# Autodesk Inventor assembly: CATFEEDER
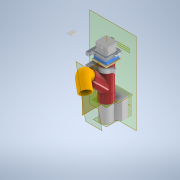
[picture p0: Inventor's stored thumbnail of the model, 180x180]
Saved by Autodesk Inventor 2020.5 (Build 245400000, 400)
## iProperties
Created: 2022-02-21
Part Number: CATFEEDER
Document SubType Name: Assembly
Designer: EDDY
Author: EDDY
## iProperties of the stored document CTF_beugel v1.ipt
Created: 2022-02-21
Part Number: CTF_beugel
Material: Generic
Document SubType Name: Modeling
Designer: Administrator
Density: 1 g/cm^3
Appearance: Default
Sending System: Autodesk Inventor 2021
Title: CTF_beugel v1
Author: Administrator
## iProperties of the stored document CTF_SUPPORTKLEMSPLITBUIS v1.ipt
Created: 2022-02-21
Part Number: CTF_SUPPORTKLEMSPLITBUIS
Material: Generic
Document SubType Name: Modeling
Designer: Administrator
Density: 1 g/cm^3
Appearance: Default
Sending System: Autodesk Inventor 2021
Title: CTF_SUPPORTKLEMSPLITBUIS v1
Author: Administrator
## iProperties of the stored document CFT_NEMA17 17HS4401 v12.ipt
Created: 2022-03-18
Part Number: CFT_NEMA17  17HS4401
Material: Generic
Document SubType Name: Modeling
Designer: Administrator
Density: 1 g/cm^3
Appearance: Default
Sending System: Autodesk Inventor 2021
Title: CFT_NEMA17 17HS4401 v12
Author: Administrator
## iProperties of the stored document CTF_MOTORFLENS v14.ipt
Created: 2022-02-21
Part Number: CTF_MOTORFLENS
Material: Generic
Document SubType Name: Modeling
Designer: Administrator
Density: 1 g/cm^3
Appearance: Default
Sending System: Autodesk Inventor 2021
Title: CTF_MOTORFLENS v14
Author: Administrator
## iProperties of the stored document CFT_arhimedes v20.ipt
Created: 2022-02-21
Part Number: CFT_arhimedes
Material: Generic
Document SubType Name: Modeling
Designer: Administrator
Density: 1 g/cm^3
Appearance: Default
Sending System: Autodesk Inventor 2021
Title: CFT_arhimedes v20
Author: Administrator
## iProperties of the stored document CTF_motortussenflens v5.ipt
Created: 2022-02-21
Part Number: CTF_motortussenflens
Material: Generic
Document SubType Name: Modeling
Designer: Administrator
Density: 1 g/cm^3
Appearance: Default
Sending System: Autodesk Inventor 2021
Title: CTF_motortussenflens v5
Author: Administrator
## iProperties of the stored document CTF_ELLEBOOG90 v6.ipt
Created: 2022-02-21
Part Number: CTF_ELLEBOOG90
Material: Generic
Document SubType Name: Modeling
Designer: Administrator
Density: 1 g/cm^3
Appearance: Default
Sending System: Autodesk Inventor 2021
Title: CTF_ELLEBOOG90 v6
Author: Administrator
## iProperties of the stored document CTF_SPLTSTUK v11.ipt
Created: 2022-02-21
Part Number: CTF_SPLTSTUK
Material: Generic
Document SubType Name: Modeling
Designer: Administrator
Density: 1 g/cm^3
Appearance: Default
Sending System: Autodesk Inventor 2021
Title: CTF_SPLTSTUK v11
Author: Administrator
## Documents named in this file (25)
- C:\IV2020_DATA\IV2020_CADFILES\Catfeeder\CATFEEDER.iam
- **C:\IV2020_DATA\IV2020_CADFILES\Catfeeder\CATFEEDER.iam*LocalDocs*xAaaaabaaAaaaaaaaAaaaa2dnAh*CTF_MOTORFLENS v14.ipt
- **C:\IV2020_DATA\IV2020_CADFILES\Catfeeder\CATFEEDER.iam*LocalDocs*xAaaaanaaAaaaaaaaAaaaqlbl5b*CTF_motortussenflens v5.ipt
- **C:\IV2020_DATA\IV2020_CADFILES\Catfeeder\CATFEEDER.iam*LocalDocs*xAaaaapaaAaaaaaaaAaaaqkmmNf*CFT_arhimedes v20.ipt
- **C:\IV2020_DATA\IV2020_CADFILES\Catfeeder\CATFEEDER.iam*LocalDocs*xAaaaqibaAaaaaaaaAaaaqnyw4c*CTF_ELLEBOOG90 v6.ipt
- **C:\IV2020_DATA\IV2020_CADFILES\Catfeeder\CATFEEDER.iam*LocalDocs*xAaaaaaaaAaaaaaaaAaaaaebq2g*CTF_SUPPORTKLEMSPLITBUIS v1.ipt
- **C:\IV2020_DATA\IV2020_CADFILES\Catfeeder\CATFEEDER.iam*LocalDocs*xAaaaahcaAaaaaaaaAaaaakzuIb*CTF_beugel v1.ipt
- **C:\IV2020_DATA\IV2020_CADFILES\Catfeeder\CATFEEDER.iam*LocalDocs*xAaaaqzbaAaaaaaaaAaaaqedeCa*CTF_SPLTSTUK v11.ipt
- C:\IV2020_DATA\IV2020_CADFILES\Imported Components\CTF_steunmotor\CTF_steunmotor.ipt
- C:\IV2020_DATA\IV2020_CADFILES\Imported Components\CFT_motorklem\CFT_motorklem.ipt
- C:\IV2020_DATA\IV2020_CADFILES\Catfeeder\CFT_kast.ipt
- C:\IV2020_DATA\IV2020_CADFILES\Catfeeder\CFT_koppelstuk.ipt
- C:\IV2020_DATA\IV2020_CADFILES\Imported Components\Stepper_Driver_WINOMO_DRV8825_RP_A4988\Stepper_Driver_WINOMO_DRV8825_RP_A4988.ipt
- **C:\IV2020_DATA\IV2020_CADFILES\Catfeeder\CATFEEDER.iam*LocalDocs*xAaaaa0caAaaaaaaaAaaaq4zbYa*CFT_NEMA17 17HS4401 v12.ipt
- C:\IV2020_DATA\IV2020_CADFILES\Catfeeder\Archimedes2schroef.ipt
- C:\IV2020_DATA\IV2020_CADFILES\Catfeeder\CTF_GOOT.ipt
- C:\IV2020_DATA\IV2020_CADFILES\Catfeeder\CTF_deksel.ipt
- C:\IV2020_DATA\IV2020_CADFILES\Catfeeder\CTF_MOTORFLENS v14.ipt
- C:\IV2020_DATA\IV2020_CADFILES\Catfeeder\CTF_motortussenflens v5.ipt
- C:\IV2020_DATA\IV2020_CADFILES\Catfeeder\CFT_arhimedes v20.ipt
- C:\IV2020_DATA\IV2020_CADFILES\Catfeeder\CTF_ELLEBOOG90 v6.ipt
- C:\IV2020_DATA\IV2020_CADFILES\Catfeeder\CTF_SUPPORTKLEMSPLITBUIS v1.ipt
- C:\IV2020_DATA\IV2020_CADFILES\Catfeeder\CTF_beugel v1.ipt
- C:\IV2020_DATA\IV2020_CADFILES\Catfeeder\CTF_SPLTSTUK v11.ipt
- C:\IV2020_DATA\IV2020_CADFILES\Catfeeder\CFT_NEMA17 17HS4401 v12.ipt
## Components (21 placed, 16 different names)
1. CTF_MOTORFLENS v14:1 — Mate:1, Mate:2, Angle:1, Mate:4, Angle:3, Angle:5, Mate:9, Mate:12, Mate:19, Flush:4
2. CTF_motortussenflens v5:1 — Mate:1, Mate:2, Angle:1, Mate:4, Insert:3, Mate:13, Mate:15, Flush:5, Mate:32
3. CFT_arhimedes v20:1 — Insert:3, Mate:31
4. CTF_ELLEBOOG90 v6:1 — Angle:3, Flush:1, Mate:18, Mate:27, Mate:28, Mate:29, Mate:30
5. CTF_ELLEBOOG90 v6:2 — Angle:6, Mate:10, Mate:11
6. CTF_SUPPORTKLEMSPLITBUIS v1:1 — Angle:5, Mate:7, Mate:8, Mate:19, Flush:3, Flush:6, Flush:7
7. CTF_beugel v1:1 — Mate:7, Mate:8
8. CTF_SPLTSTUK v11:1 — Mate:9, Angle:6, Flush:1, Mate:10, Mate:11, Mate:12, Mate:17, Mate:28, Mate:30, Flush:10, Flush:11, Flush:12, Flush:13, Flush:19, Flush:20
9. CTF_steunmotor:1 — Mate:13, Mate:15, Mate:16, Angle:7, Mate:23, Angle:8
10. CFT_motorklem:1 — Mate:16
11. CTF_SUPPORTKLEMSPLITBUIS v1:2 — Mate:17, Angle:7, Mate:20
12. CTF_SUPPORTKLEMSPLITBUIS v1:3 — Mate:18, Mate:21, Mate:22, Mate:24, Flush:6, Flush:7
13. CTF_beugel v1:2 — Mate:21, Mate:22
14. CTF_beugel v1:3 — Mate:20, Flush:9
15. CFT_kast:1 — Flush:3, Flush:4, Flush:5
16. CFT_koppelstuk:1 — Mate:27, Mate:29, Flush:9
17. Stepper_Driver_WINOMO_DRV8825_RP_A4988:1
18. CFT_NEMA17 17HS4401 v12:1 — Mate:31, Angle:10, Mate:32
19. Archimedes2schroef:1 — Flush:10, Flush:11, Flush:16, Flush:19, Flush:21
20. CTF_GOOT:1 — Flush:12, Flush:13, Flush:14, Flush:15, Flush:16, Flush:17, Flush:18, Flush:20
21. CTF_deksel:1 — Flush:14, Flush:15, Flush:17, Flush:18, Flush:21
## Relationships (57: Mate 28, Flush 20, Angle 8, Insert 1)
- Mate:1: CTF_MOTORFLENS v14:1 ↔ CTF_motortussenflens v5:1
- Mate:2: CTF_MOTORFLENS v14:1 ↔ CTF_motortussenflens v5:1
- Angle:1 (0 deg): CTF_MOTORFLENS v14:1 ↔ CTF_motortussenflens v5:1
- Mate:4: CTF_MOTORFLENS v14:1 ↔ CTF_motortussenflens v5:1
- Insert:3 (5 mm): CTF_motortussenflens v5:1 ↔ CFT_arhimedes v20:1
- Angle:3 (0 deg): CTF_MOTORFLENS v14:1 ↔ CTF_ELLEBOOG90 v6:1
- Angle:5 (0 deg): CTF_MOTORFLENS v14:1 ↔ CTF_SUPPORTKLEMSPLITBUIS v1:1
- Mate:7: CTF_SUPPORTKLEMSPLITBUIS v1:1 ↔ CTF_beugel v1:1
- Mate:8: CTF_SUPPORTKLEMSPLITBUIS v1:1 ↔ CTF_beugel v1:1
- Mate:9: CTF_MOTORFLENS v14:1 ↔ CTF_SPLTSTUK v11:1
- Angle:6 (0 deg): CTF_ELLEBOOG90 v6:2 ↔ CTF_SPLTSTUK v11:1
- Flush:1: CTF_ELLEBOOG90 v6:1 ↔ CTF_SPLTSTUK v11:1
- Mate:10: CTF_ELLEBOOG90 v6:2 ↔ CTF_SPLTSTUK v11:1
- Mate:11 (-25 mm): CTF_ELLEBOOG90 v6:2 ↔ CTF_SPLTSTUK v11:1
- Mate:12 (3 mm): CTF_MOTORFLENS v14:1 ↔ CTF_SPLTSTUK v11:1
- Mate:13: CTF_motortussenflens v5:1 ↔ CTF_steunmotor:1
- Mate:15 (2 mm): CTF_motortussenflens v5:1 ↔ CTF_steunmotor:1
- Mate:16: CTF_steunmotor:1 ↔ CFT_motorklem:1
- Mate:17: CTF_SPLTSTUK v11:1 ↔ CTF_SUPPORTKLEMSPLITBUIS v1:2
- Mate:18: CTF_ELLEBOOG90 v6:1 ↔ CTF_SUPPORTKLEMSPLITBUIS v1:3
- Angle:7 (270 deg): CTF_steunmotor:1 ↔ CTF_SUPPORTKLEMSPLITBUIS v1:2
- Mate:19: CTF_MOTORFLENS v14:1 ↔ CTF_SUPPORTKLEMSPLITBUIS v1:1
- Mate:20: CTF_SUPPORTKLEMSPLITBUIS v1:2 ↔ CTF_beugel v1:3
- Mate:21: CTF_SUPPORTKLEMSPLITBUIS v1:3 ↔ CTF_beugel v1:2
- Mate:22: CTF_SUPPORTKLEMSPLITBUIS v1:3 ↔ CTF_beugel v1:2
- Mate:23: CTF_steunmotor:1
- Mate:24: CTF_SUPPORTKLEMSPLITBUIS v1:3
- Mate:25
- Angle:8 (90 deg): CTF_steunmotor:1
- Mate:26
- Angle:9 (0 deg)
- Flush:2
- Flush:3: CTF_SUPPORTKLEMSPLITBUIS v1:1 ↔ CFT_kast:1
- Flush:4 (60 mm): CTF_MOTORFLENS v14:1 ↔ CFT_kast:1
- Flush:5 (150 mm): CTF_motortussenflens v5:1 ↔ CFT_kast:1
- Mate:27: CTF_ELLEBOOG90 v6:1 ↔ CFT_koppelstuk:1
- Flush:6: CTF_SUPPORTKLEMSPLITBUIS v1:1 ↔ CTF_SUPPORTKLEMSPLITBUIS v1:3
- Flush:7: CTF_SUPPORTKLEMSPLITBUIS v1:1 ↔ CTF_SUPPORTKLEMSPLITBUIS v1:3
- Mate:28 (-28 mm): CTF_ELLEBOOG90 v6:1 ↔ CTF_SPLTSTUK v11:1
- Mate:29: CTF_ELLEBOOG90 v6:1 ↔ CFT_koppelstuk:1
- Mate:30: CTF_ELLEBOOG90 v6:1 ↔ CTF_SPLTSTUK v11:1
- Flush:9: CTF_beugel v1:3 ↔ CFT_koppelstuk:1
- Mate:31: CFT_arhimedes v20:1 ↔ CFT_NEMA17 17HS4401 v12:1
- Angle:10 (90 deg): CFT_NEMA17 17HS4401 v12:1
- Mate:32: CTF_motortussenflens v5:1 ↔ CFT_NEMA17 17HS4401 v12:1
- Flush:10: CTF_SPLTSTUK v11:1 ↔ Archimedes2schroef:1
- Flush:11: CTF_SPLTSTUK v11:1 ↔ Archimedes2schroef:1
- Flush:12: CTF_SPLTSTUK v11:1 ↔ CTF_GOOT:1
- Flush:13: CTF_SPLTSTUK v11:1 ↔ CTF_GOOT:1
- Flush:14: CTF_GOOT:1 ↔ CTF_deksel:1
- Flush:15: CTF_GOOT:1 ↔ CTF_deksel:1
- Flush:16 (0.5 mm): Archimedes2schroef:1 ↔ CTF_GOOT:1
- Flush:17: CTF_GOOT:1 ↔ CTF_deksel:1
- Flush:18: CTF_GOOT:1 ↔ CTF_deksel:1
- Flush:19: CTF_SPLTSTUK v11:1 ↔ Archimedes2schroef:1
- Flush:20: CTF_SPLTSTUK v11:1 ↔ CTF_GOOT:1
- Flush:21: Archimedes2schroef:1 ↔ CTF_deksel:1
